# Autodesk Inventor assembly: Electromagnet final
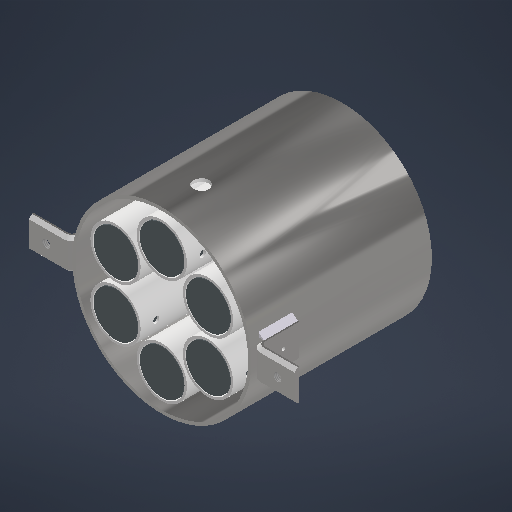
[picture p0: Inventor's stored thumbnail of the model, 512x512]
Saved by Autodesk Inventor 2026.3 (Build 303398000, 398)
## iProperties
Created: 2026-08-03
Part Number: Electromagnet final
Document SubType Name: Weldment
Designer: matot
Weld Material: Welded Aluminum-6061
Author: matot
## Documents named in this file (3)
- C:\Users\matot\OneDrive - Stellenbosch University\2026\MechatronicsProject478\Building the joint\Joint Assembly\Electromagnet final.iam
- C:\Users\matot\OneDrive - Stellenbosch University\2026\MechatronicsProject478\Building the joint\Joint Assembly\Electromagnet.iam
- C:\Users\matot\OneDrive - Stellenbosch University\2026\MechatronicsProject478\Building the joint\Joint Assembly\Pressure plate tab_L.ipt
## Components (3 placed, 2 different names)
1. Electromagnet:1 [sub-assembly] — Mate:1, Tangent:1, Mate:2, Tangent:2
2. Pressure plate tab_L:1 — Mate:2, Tangent:2
3. Pressure plate tab_L:2 — Mate:1, Tangent:1
## Relationships (4: Mate 2, Tangent 2)
- Mate:1: Electromagnet:1 ↔ Pressure plate tab_L:2
- Tangent:1: Electromagnet:1 ↔ Pressure plate tab_L:2
- Mate:2: Electromagnet:1 ↔ Pressure plate tab_L:1
- Tangent:2: Electromagnet:1 ↔ Pressure plate tab_L:1
